# Autodesk Inventor assembly: Model-4
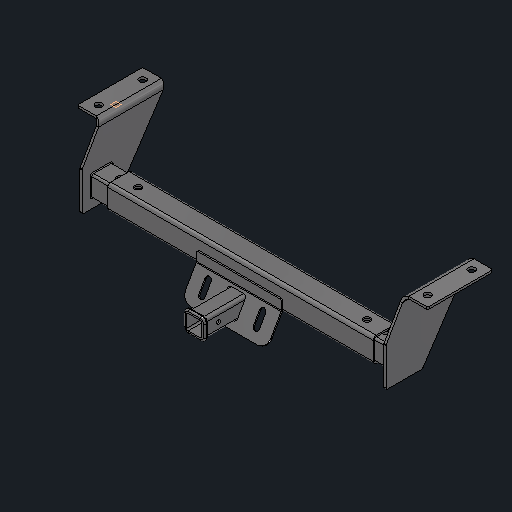
[picture p0: Inventor's stored thumbnail of the model, 512x512]
Saved by Autodesk Inventor 2025.1 (Build 291241000, 241)
## iProperties
Created: 2026-02-13
Part Number: Model-4
Document SubType Name: Assembly
Designer: Desktop -24
Mass: 20583.6 g
Surface Area: 8150.6 cm^2
Volume: 2573.11 cm^3
Density: 7.99949 g/cm^3
encoded128: ÌStandard (in)rÎ
Family: ASSEMBLY
Author: Desktop -24
## Documents named in this file (6)
- F:\OneDrive - nLeague Technologies Private Limited\Desktop\Sharath Chandra\Rear Hitch\Model-4\Model-4.iam
- F:\OneDrive - nLeague Technologies Private Limited\Desktop\Sharath Chandra\Rear Hitch\Model-4\Model-4_Sheet-LH.ipt
- F:\OneDrive - nLeague Technologies Private Limited\Desktop\Sharath Chandra\Rear Hitch\Model-4\Model-4_Sheet-RH.ipt
- F:\OneDrive - nLeague Technologies Private Limited\Desktop\Sharath Chandra\Rear Hitch\Model-4\Model-4_Base Tube-1.ipt
- F:\OneDrive - nLeague Technologies Private Limited\Desktop\Sharath Chandra\Rear Hitch\Model-4\Model-4_Sheet Stifferner.ipt
- F:\OneDrive - nLeague Technologies Private Limited\Desktop\Sharath Chandra\Rear Hitch\Model-4\Model-4_Base Tube-2.ipt
## Components (5 placed, 5 different names)
1. Model-4_Base Tube-1:1 — Mate:5, Flush:2, Mate:14, Mate:15, Mate:16, Mate:17, Mate:20, Mate:21, Mate:22, Mate:23, Flush:3, Flush:4
2. Model-4_Sheet-LH:1 — Mate:14, Mate:15, Mate:20
3. Model-4_Base Tube-2:1 — Mate:5, Flush:2, Mate:22
4. Model-4_Sheet-RH:1 — Mate:16, Mate:17, Mate:21
5. Model-4_Sheet Stifferner:1 — Mate:23, Flush:3, Flush:4
## Relationships (12: Mate 9, Flush 3)
- Mate:5: Model-4_Base Tube-1:1 ↔ Model-4_Base Tube-2:1
- Flush:2 (9.525 mm): Model-4_Base Tube-1:1 ↔ Model-4_Base Tube-2:1
- Mate:14: Model-4_Base Tube-1:1 ↔ Model-4_Sheet-LH:1
- Mate:15: Model-4_Base Tube-1:1 ↔ Model-4_Sheet-LH:1
- Mate:16: Model-4_Base Tube-1:1 ↔ Model-4_Sheet-RH:1
- Mate:17: Model-4_Base Tube-1:1 ↔ Model-4_Sheet-RH:1
- Mate:20: Model-4_Base Tube-1:1 ↔ Model-4_Sheet-LH:1
- Mate:21: Model-4_Base Tube-1:1 ↔ Model-4_Sheet-RH:1
- Mate:22: Model-4_Base Tube-1:1 ↔ Model-4_Base Tube-2:1
- Mate:23: Model-4_Base Tube-1:1 ↔ Model-4_Sheet Stifferner:1
- Flush:3 (50.8 mm): Model-4_Base Tube-1:1 ↔ Model-4_Sheet Stifferner:1
- Flush:4: Model-4_Base Tube-1:1 ↔ Model-4_Sheet Stifferner:1
